# Autodesk Inventor assembly: MicroD_MiniD_Support
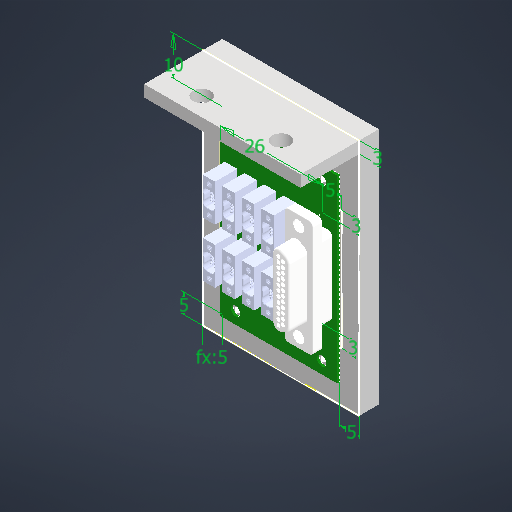
[picture p0: Inventor's stored thumbnail of the model, 512x512]
Saved by Autodesk Inventor 2026.2 (Build 302298000, 298)
## iProperties
Created: 2025-11-07
Part Number: MicroD_MiniD_Support
Document SubType Name: Assembly
Designer: alexi
Author: alexi
## Documents named in this file (3)
- C:\Jeonghyun\SNU_GIT\QSTL_Nano_D_Con_Micro_DSUB\Support\MicroD_MiniD_Support.iam
- C:\Jeonghyun\SNU_GIT\QSTL_Nano_D_Con_Micro_DSUB\Support\QSTL_Nano_D_Con_Micro_DSUB\QSTL_Nano_D_Con_Micro_DSUB.iam
- C:\Jeonghyun\SNU_GIT\QSTL_Nano_D_Con_Micro_DSUB\Support\Support.ipt
## Components (2 placed, 2 different names)
1. QSTL_Nano_D_Con_Micro_DSUB:1 [sub-assembly] — Flush:1, Flush:2
2. Support:1 — Flush:1, Flush:2
## Relationships (2: Flush 2)
- Flush:1: QSTL_Nano_D_Con_Micro_DSUB:1 ↔ Support:1
- Flush:2: QSTL_Nano_D_Con_Micro_DSUB:1 ↔ Support:1
